# Autodesk Inventor assembly: HM1_FIXT2
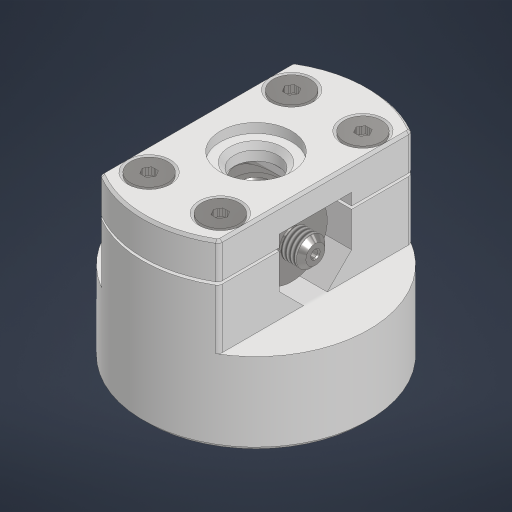
[picture p0: Inventor's stored thumbnail of the model, 512x512]
Saved by Autodesk Inventor 2024.3 (Build 283343000, 343)
## iProperties
Created: 2024-10-19
Part Number: HM1_FIXT2
Document SubType Name: Assembly
Designer: fablabadmin
Author: fablabadmin
## Documents named in this file (5)
- C:\Users\fablabadmin\Documents\_Benjamin_S\_3dCAD\HHVerkstad\Hammer1\_FIXT2\HM1_FIXT2.iam
- C:\Users\fablabadmin\Documents\_Benjamin_S\_3dCAD\HHVerkstad\Hammer1\_FIXT2\HM1_FIXT2-001.ipt
- C:\Users\fablabadmin\Documents\_Benjamin_S\_3dCAD\HHVerkstad\Hammer1\HM1-002.ipt
- C:\Users\fablabadmin\Documents\_Benjamin_S\_3dCAD\HHVerkstad\Hammer1\_FIXT2\HM1_FIXT2-002.ipt
- C:\Users\fablabadmin\Documents\Inventor\Content Center Files\R2024\en-US\ASME ANSI B18.3.5M(2)\ASME_ANSI B18.3.5M - M8x30(2).ipt
## Components (7 placed, 4 different names)
1. HM1_FIXT2-001:1 — Tangent:1, Tangent:2, Mate:1, Mate:2, Flush:1
2. HM1-002:1 — Tangent:1, Tangent:2, Mate:1, Tangent:3
3. HM1_FIXT2-002:1 — Mate:2, Flush:1, Tangent:3, Mate:3, Mate:4, Mate:5, Mate:6
4. Broached Hexagon Socket Flat Countersunk Head Cap Screws - Metric M8x30:1 — Mate:3
5. Broached Hexagon Socket Flat Countersunk Head Cap Screws - Metric M8x30:2 — Mate:4
6. Broached Hexagon Socket Flat Countersunk Head Cap Screws - Metric M8x30:3 — Mate:5
7. Broached Hexagon Socket Flat Countersunk Head Cap Screws - Metric M8x30:4 — Mate:6
## Relationships (10: Mate 6, Tangent 3, Flush 1)
- Tangent:1: HM1_FIXT2-001:1 ↔ HM1-002:1
- Tangent:2: HM1_FIXT2-001:1 ↔ HM1-002:1
- Mate:1: HM1_FIXT2-001:1 ↔ HM1-002:1
- Mate:2: HM1_FIXT2-001:1 ↔ HM1_FIXT2-002:1
- Flush:1: HM1_FIXT2-001:1 ↔ HM1_FIXT2-002:1
- Tangent:3: HM1-002:1 ↔ HM1_FIXT2-002:1
- Mate:3: HM1_FIXT2-002:1 ↔ Broached Hexagon Socket Flat Countersunk Head Cap Screws - Metric M8x30:1
- Mate:4: HM1_FIXT2-002:1 ↔ Broached Hexagon Socket Flat Countersunk Head Cap Screws - Metric M8x30:2
- Mate:5: HM1_FIXT2-002:1 ↔ Broached Hexagon Socket Flat Countersunk Head Cap Screws - Metric M8x30:3
- Mate:6: HM1_FIXT2-002:1 ↔ Broached Hexagon Socket Flat Countersunk Head Cap Screws - Metric M8x30:4
